# Autodesk Inventor assembly: Assembly_Rect_Aperture_Insert_half
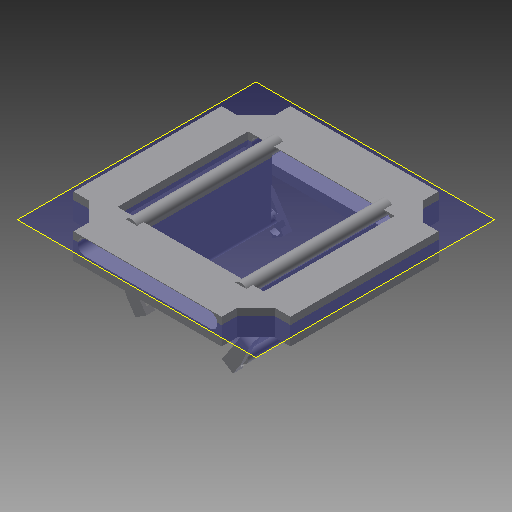
[picture p0: Inventor's stored thumbnail of the model, 512x512]
Saved by Autodesk Inventor 2019 (Build 230136000, 136)
## iProperties
Created: 2020-03-11
Part Number: Assembly_Rect_Aperture_Insert_half
Document SubType Name: Assembly
Designer: marsikovabarbora
Author: marsikovabarbora
## Documents named in this file (4)
- C:\Users\marsikovabarbora\Dropbox\UC2\02_CAD\INVENTOR\uc2_v3\Assembly_Rect_Aperture_Insert_half.iam
- C:\Users\marsikovabarbora\Dropbox\UC2\02_CAD\INVENTOR\uc2_v3\20_Rect_Aperture_Insert_half_v3.ipt
- C:\Users\marsikovabarbora\Dropbox\UC2\02_CAD\INVENTOR\uc2_v3\20_Rect_Aperture_door_hinge.ipt
- C:\Users\marsikovabarbora\Dropbox\UC2\02_CAD\INVENTOR\uc2_v3\20_Rect_Aperture_door_slide.ipt
## Components (5 placed, 3 different names)
1. 20_Rect_Aperture_Insert_half_v3:1 — Flush:1, Mate:1, Mate:2, Mate:3, Mate:4, Mate:5, Mate:6, Flush:2, Mate:7, Mate:8
2. 20_Rect_Aperture_door_hinge:1 — Mate:3, Mate:5, Mate:9
3. 20_Rect_Aperture_door_hinge:2 — Mate:4, Mate:6, Mate:10
4. 20_Rect_Aperture_door_slide:1 — Mate:7, Mate:9
5. 20_Rect_Aperture_door_slide:2 — Mate:8, Mate:10
## Relationships (12: Mate 10, Flush 2)
- Flush:1: 20_Rect_Aperture_Insert_half_v3:1
- Mate:1: 20_Rect_Aperture_Insert_half_v3:1
- Mate:2: 20_Rect_Aperture_Insert_half_v3:1
- Mate:3: 20_Rect_Aperture_Insert_half_v3:1 ↔ 20_Rect_Aperture_door_hinge:1
- Mate:4: 20_Rect_Aperture_Insert_half_v3:1 ↔ 20_Rect_Aperture_door_hinge:2
- Mate:5: 20_Rect_Aperture_Insert_half_v3:1 ↔ 20_Rect_Aperture_door_hinge:1
- Mate:6: 20_Rect_Aperture_Insert_half_v3:1 ↔ 20_Rect_Aperture_door_hinge:2
- Flush:2 (1.5 mm): 20_Rect_Aperture_Insert_half_v3:1
- Mate:7: 20_Rect_Aperture_Insert_half_v3:1 ↔ 20_Rect_Aperture_door_slide:1
- Mate:8: 20_Rect_Aperture_Insert_half_v3:1 ↔ 20_Rect_Aperture_door_slide:2
- Mate:9: 20_Rect_Aperture_door_hinge:1 ↔ 20_Rect_Aperture_door_slide:1
- Mate:10: 20_Rect_Aperture_door_hinge:2 ↔ 20_Rect_Aperture_door_slide:2
